# Autodesk Inventor assembly: ASY BSH 500 cap
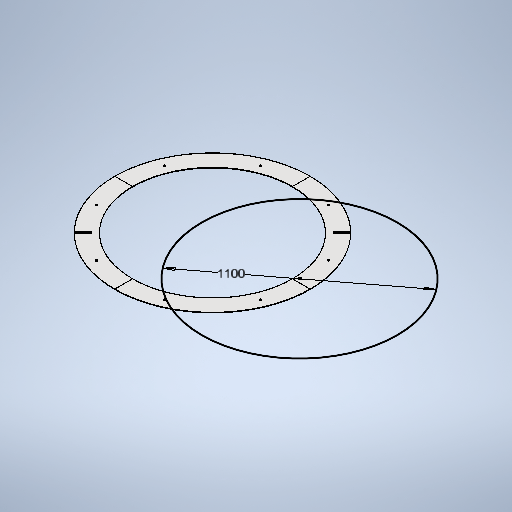
[picture p0: Inventor's stored thumbnail of the model, 512x512]
Saved by Autodesk Inventor 2025 (Build 290162010, 162A)
## iProperties
Created: 2024-09-03
Part Number: ASY BSH 500 cap
Document SubType Name: Assembly
Designer: pokla
Author: pokla
## Documents named in this file (5)
- C:\Users\pokla\Documents\Inventor\BSH_Beshkino_bio_tank\ASY BSH 500 cap.iam
- C:\Users\pokla\Documents\Inventor\BSH_Beshkino_bio_tank\BSH 501 segment.ipt
- C:\Users\pokla\Documents\Inventor\BSH_Beshkino_bio_tank\BSH 502 segment.ipt
- C:\Users\pokla\Documents\Inventor\BSH_Beshkino_bio_tank\BSH 503 inner cross.ipt
- C:\Users\pokla\Documents\Inventor\BSH_Beshkino_bio_tank\BSH DIM 500.1 parameters.ipt
## Components (6 placed, 4 different names)
1. BSH 501 segment:1 — Rigid:1
2. BSH 502 segment:1 — Rigid:1, Rigid:2
3. BSH 501 segment:2 — Rigid:2, Rigid:3
4. BSH 502 segment:2 — Rigid:3
5. BSH 503 inner cross:1
6. BSH DIM 500.1 parameters:1
## Relationships (3: WeldJoint 3)
- Rigid:1 [WeldJoint]: BSH 501 segment:1 ↔ BSH 502 segment:1
- Rigid:2 [WeldJoint]: BSH 502 segment:1 ↔ BSH 501 segment:2
- Rigid:3 [WeldJoint]: BSH 501 segment:2 ↔ BSH 502 segment:2
